# Autodesk Inventor assembly: Front A
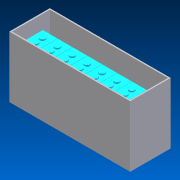
[picture p0: Inventor's stored thumbnail of the model, 180x180]
Saved by Autodesk Inventor 2012 (Build 160160000, 160)
## iProperties
Created: 2012-07-01
Part Number: Front A
Document SubType Name: Assembly
Designer: Hemant
Author: Hemant
## Documents named in this file (3)
- C:\Users\Hemant\Documents\Bat Boxes COmplete\Front A.iam
- C:\Users\Hemant\Documents\Small Battery Box Pastic 1.ipt
- C:\Users\Hemant\Documents\CALB100AH.ipt
## Components (9 placed, 2 different names)
1. Small Battery Box Pastic 1:1 — Mate:1, Mate:2, Mate:3
2. CALB100AH:1
3. CALB100AH:2
4. CALB100AH:3
5. CALB100AH:4
6. CALB100AH:5 — Mate:3
7. CALB100AH:6
8. CALB100AH:7
9. CALB100AH:8 — Mate:1, Mate:2
## Component patterns: (8 elements, first: CALB100AH:1)
## Relationships (3: Mate 3)
- Mate:1: Small Battery Box Pastic 1:1 ↔ CALB100AH:8
- Mate:2: Small Battery Box Pastic 1:1 ↔ CALB100AH:8
- Mate:3: Small Battery Box Pastic 1:1 ↔ CALB100AH:5
